# Autodesk Inventor assembly: Selection_Shaft Assy 2 Lanes
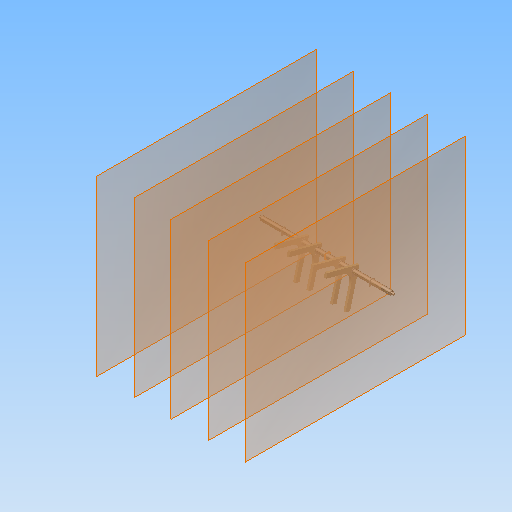
[picture p0: Inventor's stored thumbnail of the model, 512x512]
Saved by Autodesk Inventor 2018.1 (Build 221171000, 171)
## iProperties
Created: 2019-02-14
Part Number: Selection_Shaft Assy 2 Lanes
Document SubType Name: Assembly
Designer: James
Author: James
## Documents named in this file (4)
- C:\Users\admin\Desktop\Ball-Machine\Selection Sort\Selection - 2 Lanes\Selection_Shaft Assy 2 Lanes.iam
- C:\Users\admin\Desktop\Ball-Machine\Selection Sort\Selection_Selector 1.ipt
- C:\Users\admin\Desktop\Ball-Machine\Prototype CAD\Selection Sort - 40mm\BS 3673 - 6mm External Circlip.ipt
- C:\Users\admin\Desktop\Ball-Machine\Selection Sort\Selection - 2 Lanes\Selection_Shaft 1 2 Lanes.ipt
## Components (11 placed, 3 different names)
1. Selection_Shaft 1 2 Lanes:1 — Flush:1, Flush:2, Flush:3, Mate:1, Mate:2, Mate:3, Mate:4, Mate:5, Mate:6, Mate:7, Mate:8, Mate:9, Mate:10
2. BS 3673 - 6mm External Circlip:11 — Mate:7, Mate:8, Flush:8
3. BS 3673 - 6mm External Circlip:12 — Mate:9, Mate:10, Flush:7, Flush:8
4. BS 3673 - 6mm External Circlip:2 — Mate:4, Mate:5, Flush:7, Flush:9, Mate:11
5. Selection_Selector 1:1 — Mate:2, Flush:4, Mate:11
6. BS 3673 - 6mm External Circlip:1 — Mate:3, Mate:6, Flush:9, Mate:12
7. Selection_Selector 1:2 — Mate:1, Flush:4, Mate:12
8. BS 3673 - 6mm External Circlip:3
9. Selection_Selector 1:3
10. BS 3673 - 6mm External Circlip:4
11. Selection_Selector 1:4
## Component patterns: (2 elements, first: BS 3673 - 6mm External Circlip:2 + Selection_Selector 1:1 + BS 3673 - 6mm External Circlip:1 + Selection_Selector 1:2)
## Relationships (19: Mate 12, Flush 7)
- Flush:1: Selection_Shaft 1 2 Lanes:1
- Flush:2: Selection_Shaft 1 2 Lanes:1
- Flush:3: Selection_Shaft 1 2 Lanes:1
- Mate:1: Selection_Shaft 1 2 Lanes:1 ↔ Selection_Selector 1:2
- Mate:2: Selection_Shaft 1 2 Lanes:1 ↔ Selection_Selector 1:1
- Flush:4: Selection_Selector 1:1 ↔ Selection_Selector 1:2
- Mate:11: BS 3673 - 6mm External Circlip:2 ↔ Selection_Selector 1:1
- Mate:12: BS 3673 - 6mm External Circlip:1 ↔ Selection_Selector 1:2
- Mate:3: Selection_Shaft 1 2 Lanes:1 ↔ BS 3673 - 6mm External Circlip:1
- Mate:4: Selection_Shaft 1 2 Lanes:1 ↔ BS 3673 - 6mm External Circlip:2
- Mate:5: Selection_Shaft 1 2 Lanes:1 ↔ BS 3673 - 6mm External Circlip:2
- Mate:6: Selection_Shaft 1 2 Lanes:1 ↔ BS 3673 - 6mm External Circlip:1
- Mate:7: Selection_Shaft 1 2 Lanes:1 ↔ BS 3673 - 6mm External Circlip:11
- Mate:8: Selection_Shaft 1 2 Lanes:1 ↔ BS 3673 - 6mm External Circlip:11
- Mate:9: Selection_Shaft 1 2 Lanes:1 ↔ BS 3673 - 6mm External Circlip:12
- Mate:10: Selection_Shaft 1 2 Lanes:1 ↔ BS 3673 - 6mm External Circlip:12
- Flush:7: BS 3673 - 6mm External Circlip:12 ↔ BS 3673 - 6mm External Circlip:2
- Flush:8: BS 3673 - 6mm External Circlip:11 ↔ BS 3673 - 6mm External Circlip:12
- Flush:9: BS 3673 - 6mm External Circlip:2 ↔ BS 3673 - 6mm External Circlip:1
